# Autodesk Inventor assembly: CCM_Unit_C
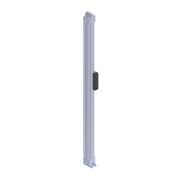
[picture p0: Inventor's stored thumbnail of the model, 180x180]
Saved by Autodesk Inventor 2020 (Build 240168000, 168)
## iProperties
Created: 2021-02-24
Part Number: CCM_Unit_C
Document SubType Name: Assembly
Designer: magnarecta
Author: magnarecta
## Documents named in this file (5)
- D:\Document\Github\Eto_Project\Hardware\Parts\CCM\CCM motion linear guide rail\CCM_UNIT\CCM_Unit_C.iam
- D:\Document\Github\Eto_Project\Hardware\Parts\CCM\CCM motion linear guide rail\CCM_UNIT\TAILSTOCK W40-00_0+0.ipt
- D:\Document\Github\Eto_Project\Hardware\Parts\CCM\CCM motion linear guide rail\CCM_UNIT\CART HK32-06W-00__1.ipt
- D:\Document\Github\Eto_Project\Hardware\Parts\CCM\CCM motion linear guide rail\CCM_UNIT\RAIL W40-06_B.ipt
- D:\Document\Github\Eto_Project\Hardware\Parts\CCM\CCM motion linear guide rail\CCM_UNIT\TAILSTOCK W40-00_0+22_1_MIR1.ipt
## Components (4 placed, 4 different names)
1. RAIL W40-06_B:1 — メイト:2, フラッシュ:3, フラッシュ:4, スライダ:1, メイト:3, フラッシュ:5, フラッシュ:6
2. TAILSTOCK W40-00_0+0:1 — メイト:2, フラッシュ:3, フラッシュ:4
3. CART HK32-06W-00__1:1 — スライダ:1
4. TAILSTOCK W40-00_0+22_1_MIR1:1 — メイト:3, フラッシュ:5, フラッシュ:6
## Relationships (7: Flush 4, Mate 2, TranslationJoint 1)
- メイト:2 [Mate]: RAIL W40-06_B:1 ↔ TAILSTOCK W40-00_0+0:1
- フラッシュ:3 [Flush]: RAIL W40-06_B:1 ↔ TAILSTOCK W40-00_0+0:1
- フラッシュ:4 [Flush]: RAIL W40-06_B:1 ↔ TAILSTOCK W40-00_0+0:1
- スライダ:1 [TranslationJoint]: RAIL W40-06_B:1 ↔ CART HK32-06W-00__1:1
- メイト:3 [Mate]: RAIL W40-06_B:1 ↔ TAILSTOCK W40-00_0+22_1_MIR1:1
- フラッシュ:5 [Flush]: RAIL W40-06_B:1 ↔ TAILSTOCK W40-00_0+22_1_MIR1:1
- フラッシュ:6 [Flush]: RAIL W40-06_B:1 ↔ TAILSTOCK W40-00_0+22_1_MIR1:1
